# Autodesk Inventor assembly: keyboard
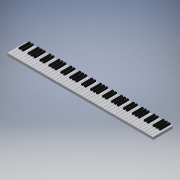
[picture p0: Inventor's stored thumbnail of the model, 180x180]
Saved by Autodesk Inventor 2017 (Build 210142000, 142)
## iProperties
Created: 2018-03-15
Part Number: keyboard
Document SubType Name: Assembly
Designer: Luiz Gustavo
Author: Luiz Gustavo
## Documents named in this file (2)
- C:\Users\Luiz Gustavo\Documents\Inventor\piano-robot\keyboard.iam
- C:\Users\Luiz Gustavo\Documents\Inventor\piano-robot\octave.iam
## Components (7 placed, 1 different names)
1. octave:1 [sub-assembly] — Flush:1, Flush:2, Flush:3, Mate:1, Mate:6
2. octave:2 [sub-assembly] — Flush:4, Flush:10, Mate:1, Mate:2
3. octave:3 [sub-assembly] — Flush:5, Flush:11, Mate:5, Mate:6
4. octave:4 [sub-assembly] — Flush:6, Flush:12, Mate:2, Mate:3
5. octave:5 [sub-assembly] — Flush:7, Flush:13, Mate:4, Mate:5
6. octave:6 [sub-assembly] — Flush:8, Flush:14, Mate:3
7. octave:7 [sub-assembly] — Flush:9, Flush:15, Mate:4
## Relationships (21: Flush 15, Mate 6)
- Flush:1: octave:1
- Flush:2: octave:1
- Flush:3: octave:1
- Flush:4: octave:2
- Flush:5: octave:3
- Flush:6: octave:4
- Flush:7: octave:5
- Flush:8: octave:6
- Flush:9: octave:7
- Flush:10: octave:2
- Flush:11: octave:3
- Flush:12: octave:4
- Flush:13: octave:5
- Flush:14: octave:6
- Flush:15: octave:7
- Mate:1: octave:1 ↔ octave:2
- Mate:2: octave:2 ↔ octave:4
- Mate:3: octave:4 ↔ octave:6
- Mate:4: octave:5 ↔ octave:7
- Mate:5: octave:3 ↔ octave:5
- Mate:6: octave:1 ↔ octave:3
